# Autodesk Inventor assembly: Whole Arm
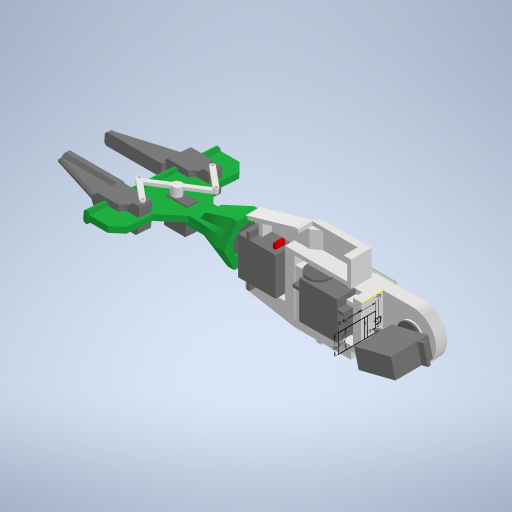
[picture p0: Inventor's stored thumbnail of the model, 512x512]
Saved by Autodesk Inventor 2023 (Build 270158000, 158)
## iProperties
Created: 2024-06-27
Part Number: Whole Arm
Document SubType Name: Assembly
Designer: Swoby
Author: Swoby
## Documents named in this file (3)
- C:\Users\Swoby\OneDrive\Plocha\DUM-E\V0.2\Whole Arm.iam
- C:\Users\Swoby\OneDrive\Plocha\DUM-E\V0.2\Gripper.iam
- C:\Users\Swoby\OneDrive\Plocha\DUM-E\V0.2\wirst.iam
## Components (2 placed, 2 different names)
1. Gripper:1 [sub-assembly] — Mate:1, Mate:2
2. wirst:1 [sub-assembly] — Mate:1, Mate:2
## Relationships (2: Mate 2)
- Mate:1: Gripper:1 ↔ wirst:1
- Mate:2: Gripper:1 ↔ wirst:1
